# Autodesk Inventor assembly: MechanumChassis
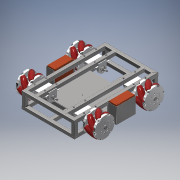
[picture p0: Inventor's stored thumbnail of the model, 180x180]
Saved by Autodesk Inventor 2018 (Build 220112000, 112)
## iProperties
Created: 2017-10-18
Part Number: MechanumChassis
Document SubType Name: Weldment
Designer: Bryce Richards
Mass: 42172.1 g
Surface Area: 44852.8 cm^2
Volume: 5448.29 cm^3
Density: 7.74044 g/cm^3
Weld Material: Steel, Mild, Welded
Author: Bryce Richards
## Documents named in this file (18)
- C:\Users\P136265\Documents\GitHub\mecanum-cad\MechanumChassis.iam
- C:\Users\P136265\Documents\GitHub\mecanum-cad\MecanumFrame2.iam
- C:\Users\P136265\Documents\GitHub\mecanum-cad\WheelShaft.ipt
- C:\Users\P136265\Documents\GitHub\mecanum-cad\Mecanum_Assembly.iam
- C:\Users\P136265\Documents\Inventor\Content Center Files\R2018\en-US\AS 1112 (2)\AS 1112 - M4  Type 5.ipt
- C:\Users\P136265\Documents\GitHub\mecanum-cad\LiftBase.ipt
- C:\Users\P136265\Documents\GitHub\mecanum-cad\BatteryBox_NP1812.ipt
- C:\Users\P136265\Documents\GitHub\mecanum-cad\NP18-12 Battery.ipt
- C:\Users\P136265\Documents\GitHub\mecanum-cad\BearingHousing.iam
- C:\Users\P136265\Documents\Inventor\Content Center Files\R2018\en-US\AS 1110\AS 1110 - M8 x 50.ipt
- C:\Users\P136265\Documents\Inventor\Content Center Files\R2018\en-US\AS 1112 (2)\AS 1112 - M8  Type 5.ipt
- C:\Users\P136265\Documents\Inventor\Content Center Files\R2018\en-US\BS EN 24035\ISO 4035 - M20BS EN.ipt
- C:\Users\P136265\Documents\mecanum-cad\MechanumChassis\AIP\FEA\cayefugld.fres
- C:\Users\P136265\Documents\mecanum-cad\MechanumChassis\AIP\FEA\cayefugao.fins
- C:\Users\P136265\Documents\mecanum-cad\MechanumChassis\AIP\FEA\cayefugao.fsat
- C:\Users\P136265\Documents\mecanum-cad\MechanumChassis\AIP\FEA\cayefugao.ftes
- C:\Users\P136265\Documents\mecanum-cad\MechanumChassis\AIP\FEA\cayefugao.fwiz
- C:\Users\P136265\Documents\mecanum-cad\MechanumChassis\AIP\FEA\cayefuglc.fmsh
## Components (66 placed, 11 different names)
1. MecanumFrame2:1 [sub-assembly] — Mate:90, Angle:5, Angle:6, Angle:7, Mate:386, Flush:32, Flush:33, Mate:486, Mate:487, Mate:488, Mate:489, Mate:494, Mate:500, Mate:501, Mate:502, Mate:503, Mate:504, Mate:512, Mate:514, Mate:516, Mate:518, Mate:520, Mate:522, Mate:524, Mate:526, Mate:528, Mate:530, Mate:532, Mate:534, Mate:536, Mate:538, Mate:540, Mate:542, Mate:545, Mate:547, Mate:549, Mate:551, Mate:553, Mate:555, Mate:557, Mate:559, Mate:561, Mate:563, Mate:565, Mate:567, Mate:569, Mate:571, Mate:573, Mate:575, Mate:594
2. Mecanum_Assembly:1 [sub-assembly] — Mate:318, Mate:319, Flush:28, Mate:602
3. Mecanum_Assembly:2 [sub-assembly] — Mate:498, Mate:499, Angle:34, Mate:600
4. Mecanum_Assembly:3 [sub-assembly] — Mate:507, Mate:508, Angle:35, Mate:598
5. Mecanum_Assembly:4 [sub-assembly] — Mate:592, Angle:39, Mate:593, Mate:596
6. WheelShaft:1 — Mate:490, Mate:491, Mate:492, Mate:586, Mate:592, Angle:39, Mate:593, Mate:595
7. WheelShaft:2 — Mate:318, Mate:319, Flush:28, Mate:509, Mate:510, Mate:588, Mate:601
8. WheelShaft:3 — Mate:505, Mate:506, Mate:507, Mate:508, Angle:35, Mate:590, Mate:597
9. WheelShaft:4 — Mate:492, Mate:497, Mate:498, Mate:499, Angle:34, Mate:584, Mate:599
10. LiftBase:1 — Mate:386, Flush:32, Flush:33
11. BatteryBox_NP1812:1 — Mate:459, Mate:461
12. BatteryBox_NP1812:2 — Mate:462, Mate:464
13. NP18-12 Battery:1 — Mate:459, Mate:461
14. NP18-12 Battery:2 — Mate:462, Mate:464
15. AS 1112 (2) - Metric M4  Type 5:17
16. AS 1112 (2) - Metric M4  Type 5:18
17. AS 1112 (2) - Metric M4  Type 5:19
18. AS 1112 (2) - Metric M4  Type 5:20
19. AS 1112 (2) - Metric M4  Type 5:21
20. AS 1112 (2) - Metric M4  Type 5:22
21. AS 1112 (2) - Metric M4  Type 5:23
22. AS 1112 (2) - Metric M4  Type 5:24
23. BearingHousing:1 [sub-assembly] — Mate:486, Mate:487, Mate:488, Mate:489, Mate:490, Mate:491, Mate:493, Mate:521, Mate:523, Mate:525, Mate:527, Mate:587
24. BearingHousing:2 [sub-assembly] — Mate:493, Mate:494, Mate:497, Mate:513, Mate:515, Mate:517, Mate:519, Mate:585, Mate:594
25. BearingHousing:3 [sub-assembly] — Mate:503, Mate:504, Mate:505, Mate:506, Mate:529, Mate:531, Mate:533, Mate:535, Mate:591
26. BearingHousing:4 [sub-assembly] — Mate:500, Mate:501, Mate:502, Mate:509, Mate:510, Mate:537, Mate:539, Mate:541, Mate:543, Mate:589
27. AS 1110 - Metric M8 x 50:3 — Mate:512, Mate:513, Mate:558
28. AS 1110 - Metric M8 x 50:4 — Mate:514, Mate:515, Mate:556
29. AS 1110 - Metric M8 x 50:5 — Mate:516, Mate:517, Mate:552
30. AS 1110 - Metric M8 x 50:6 — Mate:518, Mate:519, Mate:554
31. AS 1110 - Metric M8 x 50:7 — Mate:520, Mate:521, Mate:574
32. AS 1110 - Metric M8 x 50:8 — Mate:522, Mate:523, Mate:572
33. AS 1110 - Metric M8 x 50:9 — Mate:524, Mate:525, Mate:568
34. AS 1110 - Metric M8 x 50:10 — Mate:526, Mate:527, Mate:570
35. AS 1110 - Metric M8 x 50:11 — Mate:528, Mate:529, Mate:566
36. AS 1110 - Metric M8 x 50:12 — Mate:530, Mate:531, Mate:562
37. AS 1110 - Metric M8 x 50:13 — Mate:532, Mate:533, Mate:564
38. AS 1110 - Metric M8 x 50:14 — Mate:534, Mate:535, Mate:560
39. AS 1110 - Metric M8 x 50:15 — Mate:536, Mate:537, Mate:544
40. AS 1110 - Metric M8 x 50:16 — Mate:538, Mate:539, Mate:548
41. AS 1110 - Metric M8 x 50:17 — Mate:540, Mate:541, Mate:546
42. AS 1110 - Metric M8 x 50:18 — Mate:542, Mate:543, Mate:550
43. AS 1112 (2) - Metric M8  Type 5:1 — Mate:544, Mate:545
44. AS 1112 (2) - Metric M8  Type 5:2 — Mate:546, Mate:547
45. AS 1112 (2) - Metric M8  Type 5:3 — Mate:548, Mate:549
46. AS 1112 (2) - Metric M8  Type 5:4 — Mate:550, Mate:551
47. AS 1112 (2) - Metric M8  Type 5:5 — Mate:552, Mate:553
48. AS 1112 (2) - Metric M8  Type 5:6 — Mate:554, Mate:555
49. AS 1112 (2) - Metric M8  Type 5:7 — Mate:556, Mate:557
50. AS 1112 (2) - Metric M8  Type 5:8 — Mate:558, Mate:559
51. AS 1112 (2) - Metric M8  Type 5:9 — Mate:560, Mate:561
52. AS 1112 (2) - Metric M8  Type 5:10 — Mate:562, Mate:563
53. AS 1112 (2) - Metric M8  Type 5:11 — Mate:564, Mate:565
54. AS 1112 (2) - Metric M8  Type 5:12 — Mate:566, Mate:567
55. AS 1112 (2) - Metric M8  Type 5:13 — Mate:568, Mate:569
56. AS 1112 (2) - Metric M8  Type 5:14 — Mate:570, Mate:571
57. AS 1112 (2) - Metric M8  Type 5:15 — Mate:572, Mate:573
58. AS 1112 (2) - Metric M8  Type 5:16 — Mate:574, Mate:575
59. BS EN 24035 - Metric M20:5 — Mate:584, Mate:585
60. BS EN 24035 - Metric M20:6 — Mate:586, Mate:587
61. BS EN 24035 - Metric M20:7 — Mate:588, Mate:589
62. BS EN 24035 - Metric M20:8 — Mate:590, Mate:591
63. BS EN 24035 - Metric M20:9 — Mate:595, Mate:596
64. BS EN 24035 - Metric M20:10 — Mate:597, Mate:598
65. BS EN 24035 - Metric M20:11 — Mate:599, Mate:600
66. BS EN 24035 - Metric M20:12 — Mate:601, Mate:602
## Relationships (123: Mate 114, Angle 6, Flush 3)
- Mate:90: MecanumFrame2:1
- Angle:5 (0 deg): MecanumFrame2:1
- Angle:6 (0 deg): MecanumFrame2:1
- Angle:7 (0 deg): MecanumFrame2:1
- Mate:318: Mecanum_Assembly:1 ↔ WheelShaft:2
- Mate:319: Mecanum_Assembly:1 ↔ WheelShaft:2
- Flush:28: Mecanum_Assembly:1 ↔ WheelShaft:2
- Mate:386: MecanumFrame2:1 ↔ LiftBase:1
- Flush:32 (2.5 mm): MecanumFrame2:1 ↔ LiftBase:1
- Flush:33 (2.5 mm): MecanumFrame2:1 ↔ LiftBase:1
- Mate:459: BatteryBox_NP1812:1 ↔ NP18-12 Battery:1
- Mate:461 (2 mm): BatteryBox_NP1812:1 ↔ NP18-12 Battery:1
- Mate:462: BatteryBox_NP1812:2 ↔ NP18-12 Battery:2
- Mate:464 (2 mm): BatteryBox_NP1812:2 ↔ NP18-12 Battery:2
- Mate:486: MecanumFrame2:1 ↔ BearingHousing:1
- Mate:487: MecanumFrame2:1 ↔ BearingHousing:1
- Mate:488: MecanumFrame2:1 ↔ BearingHousing:1
- Mate:489: MecanumFrame2:1 ↔ BearingHousing:1
- Mate:490: WheelShaft:1 ↔ BearingHousing:1
- Mate:491: WheelShaft:1 ↔ BearingHousing:1
- Mate:492: WheelShaft:1 ↔ WheelShaft:4
- Mate:493: BearingHousing:1 ↔ BearingHousing:2
- Mate:494: MecanumFrame2:1 ↔ BearingHousing:2
- Mate:497: WheelShaft:4 ↔ BearingHousing:2
- Mate:498: Mecanum_Assembly:2 ↔ WheelShaft:4
- Mate:499: Mecanum_Assembly:2 ↔ WheelShaft:4
- Angle:34 (0 deg): Mecanum_Assembly:2 ↔ WheelShaft:4
- Mate:500: MecanumFrame2:1 ↔ BearingHousing:4
- Mate:501: MecanumFrame2:1 ↔ BearingHousing:4
- Mate:502: MecanumFrame2:1 ↔ BearingHousing:4
- Mate:503: MecanumFrame2:1 ↔ BearingHousing:3
- Mate:504: MecanumFrame2:1 ↔ BearingHousing:3
- Mate:505: WheelShaft:3 ↔ BearingHousing:3
- Mate:506: WheelShaft:3 ↔ BearingHousing:3
- Mate:507: Mecanum_Assembly:3 ↔ WheelShaft:3
- Mate:508: Mecanum_Assembly:3 ↔ WheelShaft:3
- Angle:35 (0 deg): Mecanum_Assembly:3 ↔ WheelShaft:3
- Mate:509: WheelShaft:2 ↔ BearingHousing:4
- Mate:510: WheelShaft:2 ↔ BearingHousing:4
- Mate:512: MecanumFrame2:1 ↔ AS 1110 - Metric M8 x 50:3
- Mate:513: BearingHousing:2 ↔ AS 1110 - Metric M8 x 50:3
- Mate:514: MecanumFrame2:1 ↔ AS 1110 - Metric M8 x 50:4
- Mate:515: BearingHousing:2 ↔ AS 1110 - Metric M8 x 50:4
- Mate:516: MecanumFrame2:1 ↔ AS 1110 - Metric M8 x 50:5
- Mate:517: BearingHousing:2 ↔ AS 1110 - Metric M8 x 50:5
- Mate:518: MecanumFrame2:1 ↔ AS 1110 - Metric M8 x 50:6
- Mate:519: BearingHousing:2 ↔ AS 1110 - Metric M8 x 50:6
- Mate:520: MecanumFrame2:1 ↔ AS 1110 - Metric M8 x 50:7
- Mate:521: BearingHousing:1 ↔ AS 1110 - Metric M8 x 50:7
- Mate:522: MecanumFrame2:1 ↔ AS 1110 - Metric M8 x 50:8
- Mate:523: BearingHousing:1 ↔ AS 1110 - Metric M8 x 50:8
- Mate:524: MecanumFrame2:1 ↔ AS 1110 - Metric M8 x 50:9
- Mate:525: BearingHousing:1 ↔ AS 1110 - Metric M8 x 50:9
- Mate:526: MecanumFrame2:1 ↔ AS 1110 - Metric M8 x 50:10
- Mate:527: BearingHousing:1 ↔ AS 1110 - Metric M8 x 50:10
- Mate:528: MecanumFrame2:1 ↔ AS 1110 - Metric M8 x 50:11
- Mate:529: BearingHousing:3 ↔ AS 1110 - Metric M8 x 50:11
- Mate:530: MecanumFrame2:1 ↔ AS 1110 - Metric M8 x 50:12
- Mate:531: BearingHousing:3 ↔ AS 1110 - Metric M8 x 50:12
- Mate:532: MecanumFrame2:1 ↔ AS 1110 - Metric M8 x 50:13
- Mate:533: BearingHousing:3 ↔ AS 1110 - Metric M8 x 50:13
- Mate:534: MecanumFrame2:1 ↔ AS 1110 - Metric M8 x 50:14
- Mate:535: BearingHousing:3 ↔ AS 1110 - Metric M8 x 50:14
- Mate:536: MecanumFrame2:1 ↔ AS 1110 - Metric M8 x 50:15
- Mate:537: BearingHousing:4 ↔ AS 1110 - Metric M8 x 50:15
- Mate:538: MecanumFrame2:1 ↔ AS 1110 - Metric M8 x 50:16
- Mate:539: BearingHousing:4 ↔ AS 1110 - Metric M8 x 50:16
- Mate:540: MecanumFrame2:1 ↔ AS 1110 - Metric M8 x 50:17
- Mate:541: BearingHousing:4 ↔ AS 1110 - Metric M8 x 50:17
- Mate:542: MecanumFrame2:1 ↔ AS 1110 - Metric M8 x 50:18
- Mate:543: BearingHousing:4 ↔ AS 1110 - Metric M8 x 50:18
- Mate:544: AS 1110 - Metric M8 x 50:15 ↔ AS 1112 (2) - Metric M8  Type 5:1
- Mate:545: MecanumFrame2:1 ↔ AS 1112 (2) - Metric M8  Type 5:1
- Mate:546: AS 1110 - Metric M8 x 50:17 ↔ AS 1112 (2) - Metric M8  Type 5:2
- Mate:547: MecanumFrame2:1 ↔ AS 1112 (2) - Metric M8  Type 5:2
- Mate:548: AS 1110 - Metric M8 x 50:16 ↔ AS 1112 (2) - Metric M8  Type 5:3
- Mate:549: MecanumFrame2:1 ↔ AS 1112 (2) - Metric M8  Type 5:3
- Mate:550: AS 1110 - Metric M8 x 50:18 ↔ AS 1112 (2) - Metric M8  Type 5:4
- Mate:551: MecanumFrame2:1 ↔ AS 1112 (2) - Metric M8  Type 5:4
- Mate:552: AS 1110 - Metric M8 x 50:5 ↔ AS 1112 (2) - Metric M8  Type 5:5
- Mate:553: MecanumFrame2:1 ↔ AS 1112 (2) - Metric M8  Type 5:5
- Mate:554: AS 1110 - Metric M8 x 50:6 ↔ AS 1112 (2) - Metric M8  Type 5:6
- Mate:555: MecanumFrame2:1 ↔ AS 1112 (2) - Metric M8  Type 5:6
- Mate:556: AS 1110 - Metric M8 x 50:4 ↔ AS 1112 (2) - Metric M8  Type 5:7
- Mate:557: MecanumFrame2:1 ↔ AS 1112 (2) - Metric M8  Type 5:7
- Mate:558: AS 1110 - Metric M8 x 50:3 ↔ AS 1112 (2) - Metric M8  Type 5:8
- Mate:559: MecanumFrame2:1 ↔ AS 1112 (2) - Metric M8  Type 5:8
- Mate:560: AS 1110 - Metric M8 x 50:14 ↔ AS 1112 (2) - Metric M8  Type 5:9
- Mate:561: MecanumFrame2:1 ↔ AS 1112 (2) - Metric M8  Type 5:9
- Mate:562: AS 1110 - Metric M8 x 50:12 ↔ AS 1112 (2) - Metric M8  Type 5:10
- Mate:563: MecanumFrame2:1 ↔ AS 1112 (2) - Metric M8  Type 5:10
- Mate:564: AS 1110 - Metric M8 x 50:13 ↔ AS 1112 (2) - Metric M8  Type 5:11
- Mate:565: MecanumFrame2:1 ↔ AS 1112 (2) - Metric M8  Type 5:11
- Mate:566: AS 1110 - Metric M8 x 50:11 ↔ AS 1112 (2) - Metric M8  Type 5:12
- Mate:567: MecanumFrame2:1 ↔ AS 1112 (2) - Metric M8  Type 5:12
- Mate:568: AS 1110 - Metric M8 x 50:9 ↔ AS 1112 (2) - Metric M8  Type 5:13
- Mate:569: MecanumFrame2:1 ↔ AS 1112 (2) - Metric M8  Type 5:13
- Mate:570: AS 1110 - Metric M8 x 50:10 ↔ AS 1112 (2) - Metric M8  Type 5:14
- Mate:571: MecanumFrame2:1 ↔ AS 1112 (2) - Metric M8  Type 5:14
- Mate:572: AS 1110 - Metric M8 x 50:8 ↔ AS 1112 (2) - Metric M8  Type 5:15
- Mate:573: MecanumFrame2:1 ↔ AS 1112 (2) - Metric M8  Type 5:15
- Mate:574: AS 1110 - Metric M8 x 50:7 ↔ AS 1112 (2) - Metric M8  Type 5:16
- Mate:575: MecanumFrame2:1 ↔ AS 1112 (2) - Metric M8  Type 5:16
- Mate:584: WheelShaft:4 ↔ BS EN 24035 - Metric M20:5
- Mate:585: BearingHousing:2 ↔ BS EN 24035 - Metric M20:5
- Mate:586: WheelShaft:1 ↔ BS EN 24035 - Metric M20:6
- Mate:587: BearingHousing:1 ↔ BS EN 24035 - Metric M20:6
- Mate:588: WheelShaft:2 ↔ BS EN 24035 - Metric M20:7
- Mate:589: BearingHousing:4 ↔ BS EN 24035 - Metric M20:7
- Mate:590: WheelShaft:3 ↔ BS EN 24035 - Metric M20:8
- Mate:591: BearingHousing:3 ↔ BS EN 24035 - Metric M20:8
- Mate:592: Mecanum_Assembly:4 ↔ WheelShaft:1
- Angle:39 (0 deg): Mecanum_Assembly:4 ↔ WheelShaft:1
- Mate:593: Mecanum_Assembly:4 ↔ WheelShaft:1
- Mate:594: MecanumFrame2:1 ↔ BearingHousing:2
- Mate:595: WheelShaft:1 ↔ BS EN 24035 - Metric M20:9
- Mate:596: Mecanum_Assembly:4 ↔ BS EN 24035 - Metric M20:9
- Mate:597: WheelShaft:3 ↔ BS EN 24035 - Metric M20:10
- Mate:598: Mecanum_Assembly:3 ↔ BS EN 24035 - Metric M20:10
- Mate:599: WheelShaft:4 ↔ BS EN 24035 - Metric M20:11
- Mate:600: Mecanum_Assembly:2 ↔ BS EN 24035 - Metric M20:11
- Mate:601: WheelShaft:2 ↔ BS EN 24035 - Metric M20:12
- Mate:602: Mecanum_Assembly:1 ↔ BS EN 24035 - Metric M20:12
## Named parameters: sa_0 = 0, sa_1 = -3.88819e-08, sa_2 = 1e+06
note: some values were not read from the file. Shown as the stored number, unit unknown: "sa_0", "sa_1", "sa_2".
